# Autodesk Inventor assembly: Rover
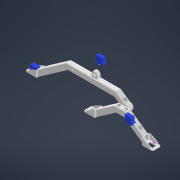
[picture p0: Inventor's stored thumbnail of the model, 180x180]
Saved by Autodesk Inventor 2021 (Build 250183000, 183)
## iProperties
Created: 2021-01-03
Part Number: Rover
Document SubType Name: Assembly
Designer: laure
Author: laure
## Documents named in this file (6)
- E:\Projects\Rover\Rover.iam
- E:\Projects\Rover\Rocker_hinten.ipt
- E:\Projects\Rover\Rocker_vorne.ipt
- E:\Projects\Rover\Bogie.ipt
- E:\Projects\Rover\Servohalterung.ipt
- E:\Projects\Rover\MicroServo.ipt
## Components (9 placed, 5 different names)
1. Fahrwerk_rocker_hinten:1 — Fluchtend:1, Fluchtend:2, Fluchtend:3, Passend:1, Passend:2, Passend:3, Winkel:1
2. Fahrwerk_rocker_vorne:1 — Fluchtend:1, Fluchtend:2, Fluchtend:3, Passend:1, Fluchtend:4, Fluchtend:5, Fluchtend:6, Passend:4
3. Fahrwerk_bogie:1 — Passend:2, Passend:3, Winkel:1, Fluchtend:7, Fluchtend:8, Fluchtend:9, Passend:5, Fluchtend:10, Fluchtend:11, Fluchtend:12, Passend:6
4. Servohalterung:1 — Fluchtend:4, Fluchtend:5, Fluchtend:6, Passend:4, Passend:7, Passend:8, Passend:9
5. Servohalterung:2 — Fluchtend:7, Fluchtend:8, Fluchtend:9, Passend:5
6. Servohalterung:3 — Fluchtend:10, Fluchtend:11, Fluchtend:12, Passend:6
7. MicroServo:1 — Passend:7, Passend:8, Passend:9
8. MicroServo:2
9. MicroServo:3
## Relationships (22: Flush 12, Mate 9, Angle 1)
- Fluchtend:1 [Flush]: Fahrwerk_rocker_hinten:1 ↔ Fahrwerk_rocker_vorne:1
- Fluchtend:2 [Flush]: Fahrwerk_rocker_hinten:1 ↔ Fahrwerk_rocker_vorne:1
- Fluchtend:3 [Flush]: Fahrwerk_rocker_hinten:1 ↔ Fahrwerk_rocker_vorne:1
- Passend:1 [Mate]: Fahrwerk_rocker_hinten:1 ↔ Fahrwerk_rocker_vorne:1
- Passend:2 [Mate]: Fahrwerk_rocker_hinten:1 ↔ Fahrwerk_bogie:1
- Passend:3 [Mate]: Fahrwerk_rocker_hinten:1 ↔ Fahrwerk_bogie:1
- Winkel:1 [Angle] (0 deg): Fahrwerk_rocker_hinten:1 ↔ Fahrwerk_bogie:1
- Fluchtend:4 [Flush]: Fahrwerk_rocker_vorne:1 ↔ Servohalterung:1
- Fluchtend:5 [Flush]: Fahrwerk_rocker_vorne:1 ↔ Servohalterung:1
- Fluchtend:6 [Flush]: Fahrwerk_rocker_vorne:1 ↔ Servohalterung:1
- Passend:4 [Mate]: Fahrwerk_rocker_vorne:1 ↔ Servohalterung:1
- Fluchtend:7 [Flush]: Fahrwerk_bogie:1 ↔ Servohalterung:2
- Fluchtend:8 [Flush]: Fahrwerk_bogie:1 ↔ Servohalterung:2
- Fluchtend:9 [Flush]: Fahrwerk_bogie:1 ↔ Servohalterung:2
- Passend:5 [Mate]: Fahrwerk_bogie:1 ↔ Servohalterung:2
- Fluchtend:10 [Flush]: Fahrwerk_bogie:1 ↔ Servohalterung:3
- Fluchtend:11 [Flush]: Fahrwerk_bogie:1 ↔ Servohalterung:3
- Fluchtend:12 [Flush]: Fahrwerk_bogie:1 ↔ Servohalterung:3
- Passend:6 [Mate]: Fahrwerk_bogie:1 ↔ Servohalterung:3
- Passend:7 [Mate] (0.75 mm): Servohalterung:1 ↔ MicroServo:1
- Passend:8 [Mate] (0.25 mm): Servohalterung:1 ↔ MicroServo:1
- Passend:9 [Mate]: Servohalterung:1 ↔ MicroServo:1
